# Autodesk Inventor assembly: アームアセンブリ
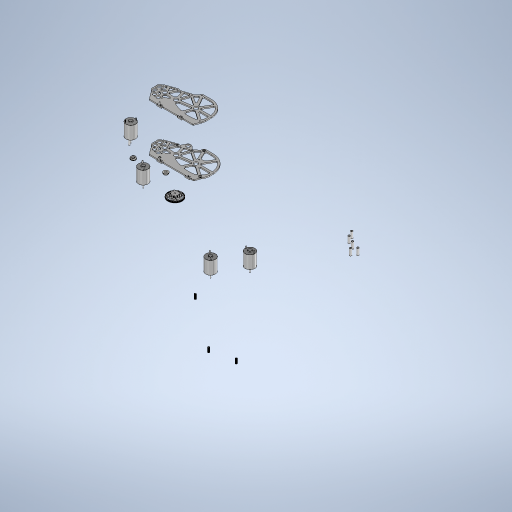
[picture p0: Inventor's stored thumbnail of the model, 512x512]
Saved by Autodesk Inventor 2023 (Build 270158000, 158)
## iProperties
Created: 2022-03-06
Part Number: アームアセンブリ
Document SubType Name: Assembly
Designer: acps
Author: acps
## Documents named in this file (9)
- C:\Users\acps\Documents\srdc\srdc_ksh\アーム\アームアセンブリ.iam
- C:\Users\acps\Documents\srdc\srdc_ksh\アーム\ギア\初段_多段ギア.iam
- C:\Users\acps\Documents\srdc\srdc_ksh\モータ\M-RS-380.ipt
- C:\Users\acps\Documents\srdc\srdc_ksh\アーム\ギアマウント.ipt
- C:\Users\acps\Documents\srdc\srdc_ksh\アーム\ギア\ぴにょん.ipt
- C:\Users\acps\Documents\srdc\srdc_ksh\ベアリング\φ6φ12ベアリングa.ipt
- C:\Users\acps\Documents\srdc\srdc_ksh\アーム\ギアマウント2.ipt
- C:\Users\acps\Documents\srdc\srdc_ksh\ピン\φ4l25.ipt
- C:\Users\acps\Documents\srdc\srdc_ksh\スペーサ\l18.ipt
## Components (18 placed, 8 different names)
1. M-RS-380:1
2. M-RS-380:2
3. ぴにょん:2
4. ぴにょん:3
5. ぴにょん:4
6. ギアマウント:2 — Mate:1, Mate:2
7. ギアマウント2:1 — Mate:1, Mate:2
8. M-RS-380:3
9. M-RS-380:4
10. 初段_多段ギア:1 [sub-assembly]
11. φ6φ12ベアリングa:1
12. φ6φ12ベアリングa:2
13. φ4l25:1
14. l18:1
15. l18:2
16. l18:3
17. l18:4
18. l18:5
## Relationships (2: Mate 2)
- Mate:1: ギアマウント:2 ↔ ギアマウント2:1
- Mate:2: ギアマウント:2 ↔ ギアマウント2:1
